# Autodesk Inventor assembly: Ratchet
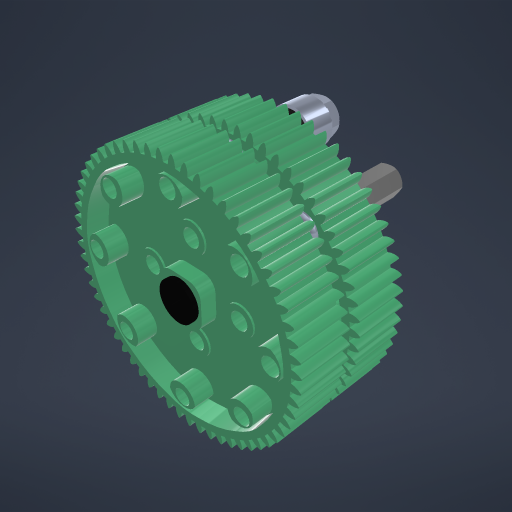
[picture p0: Inventor's stored thumbnail of the model, 512x512]
Saved by Autodesk Inventor 2023 (Build 270158000, 158)
## iProperties
Created: 2022-11-12
Part Number: Ratchet
Document SubType Name: Assembly
Designer: alex
Author: alex
## Documents named in this file (16)
- C:\Users\alex\Documents\GitHub\4067X_spin_up_cad\Ratchet.iam
- C:\Users\alex\Documents\GitHub\4067X_spin_up_cad\Library\Motion\Gears\HS 60T Gear, Circle.ipt
- C:\Users\alex\Documents\GitHub\4067X_spin_up_cad\Library\Motion\Sprockets\HS 6T Sprocket, Square.ipt
- C:\Users\alex\Documents\GitHub\4067X_spin_up_cad\Library\Motion\Spacers\Spacer Nylon .375 OD.ipt
- C:\Users\alex\Documents\GitHub\4067X_spin_up_cad\Library\Motion\Spacers\Washer Teflon.ipt
- C:\Users\alex\Documents\GitHub\4067X_spin_up_cad\Library\Structure\Hardware\Screw Steel - Star.ipt
- C:\Users\alex\Documents\GitHub\4067X_spin_up_cad\Library\Structure\Hardware\Nut Thin Nylock.ipt
- C:\Users\alex\Documents\GitHub\4067X_spin_up_cad\Library\Motion\Spacers\Spacer Nylon .375 OD\NSpacer .375 OD x .125.ipt
- C:\Users\alex\Documents\GitHub\4067X_spin_up_cad\Library\Motion\Shaft Collar without Set Screw.ipt
- C:\Users\alex\Documents\GitHub\4067X_spin_up_cad\Library\Motion\Spacers\Washer Teflon\TWasher .375 OD x .06250.ipt
- C:\Users\alex\Documents\GitHub\4067X_spin_up_cad\Library\Structure\Hardware\Screw Steel - Star\SScrew Star Smooth .625.ipt
- C:\Users\alex\Documents\GitHub\4067X_spin_up_cad\Library\Structure\Standoff\Standoff .50.ipt
- C:\Users\alex\Documents\GitHub\4067X_spin_up_cad\Library\Structure\Standoff.ipt
- C:\Users\alex\Documents\GitHub\4067X_spin_up_cad\Library\Structure\Hardware\Screw Steel - Star\SScrew Star Smooth 1.000.ipt
- C:\Users\alex\Documents\GitHub\4067X_spin_up_cad\Library\Structure\Hardware\Nut Keps.ipt
- C:\Users\alex\Documents\GitHub\4067X_spin_up_cad\Library\Motion\Gears\HS 60T Gear, Square.ipt
## Components (14 placed, 11 different names)
1. HS 60T Gear, Circle:1 — Insert:24, Insert:25, Insert:28
2. HS 6T Sprocket, Square:1
3. Nut Thin Nylock:1
4. Nut Thin Nylock:2
5. NSpacer .375 OD x .125:3 — Insert:29
6. Shaft Collar without Set Screw:1 — Insert:29, Insert:30
7. SScrew Star Smooth .625:3
8. Standoff .50:1
9. SScrew Star Smooth 1.000:5 — Insert:24
10. TWasher .375 OD x .06250:5 — Insert:25, Insert:26
11. TWasher .375 OD x .06250:6 — Insert:26, Insert:31
12. SScrew Star Smooth 1.000:6 — Insert:28
13. Nut Keps:1 — Insert:30
14. HS 60T Gear, Square:1 — Insert:31
## Relationships (13: Insert 12, Mate 1)
- [Insert]: HS 60T Gear, Circle:1 ↔ Nut Thin Nylock:1
- [Insert]: HS 60T Gear, Circle:1 ↔ Nut Thin Nylock:2
- [Insert]: HS 60T Gear, Circle:1 ↔ NSpacer .375 OD x .125:3
- [Insert]: HS 60T Gear, Circle:1 ↔ HS 6T Sprocket, Square:1
- [Mate]: Shaft Collar without Set Screw:1 ↔ SScrew Star Smooth .625:3
- [Insert]: HS 60T Gear, Circle:1 ↔ Standoff .50:1
- Insert:24: HS 60T Gear, Circle:1 ↔ SScrew Star Smooth 1.000:5
- Insert:25: HS 60T Gear, Circle:1 ↔ TWasher .375 OD x .06250:5
- Insert:26: TWasher .375 OD x .06250:5 ↔ TWasher .375 OD x .06250:6
- Insert:28: HS 60T Gear, Circle:1 ↔ SScrew Star Smooth 1.000:6
- Insert:29: NSpacer .375 OD x .125:3 ↔ Shaft Collar without Set Screw:1
- Insert:30: Shaft Collar without Set Screw:1 ↔ Nut Keps:1
- Insert:31: TWasher .375 OD x .06250:6 ↔ HS 60T Gear, Square:1
## Named parameters: d8_d9 = 0 mm, d10_d17 = 0 mm
